# Autodesk Inventor assembly: Lidar Sensor Lexan Assembly
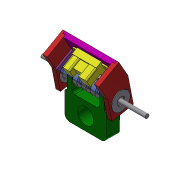
[picture p0: Inventor's stored thumbnail of the model, 180x180]
Saved by Autodesk Inventor 2018.3 (Build 223284000, 284)
## iProperties
Created: 2019-02-26
Part Number: Lidar Sensor Lexan Assembly
Document SubType Name: Assembly
Designer: aye06091
Mass: 65.9637 g
Surface Area: 342.343 cm^2
Volume: 65.9637 cm^3
Density: 1 g/cm^3
Author: aye06091
## Documents named in this file (10)
- Y:\DeSimony-R\Senior R&D\4 R&D Shared Folder\VisiStick\VisiStick (Inventor)\Case Final\Lidar Sensor Lexan Assembly.iam
- Y:\DeSimony-R\Senior R&D\4 R&D Shared Folder\VisiStick\VisiStick (Inventor)\Case Final\Lidar Sensor CAse Piece 1.ipt
- Y:\DeSimony-R\Senior R&D\4 R&D Shared Folder\VisiStick\VisiStick (Inventor)\Case Final\Lidar Sensor Case Piece 2.ipt
- Y:\DeSimony-R\Senior R&D\4 R&D Shared Folder\VisiStick\VisiStick (Inventor)\Case Final\Lidar Sensor Case Piece 3.ipt
- Y:\DeSimony-R\Senior R&D\4 R&D Shared Folder\VisiStick\VisiStick (Inventor)\Electronics\Sharp 2Y0A02.ipt
- Y:\DeSimony-R\Senior R&D\4 R&D Shared Folder\VisiStick\VisiStick (Inventor)\Physical Parts\Lidar Sensor Case 4 v2.ipt
- Y:\DeSimony-R\Senior R&D\4 R&D Shared Folder\VisiStick\VisiStick (Inventor)\Case Final\Ball Bearing.ipt
- Y:\DeSimony-R\Senior R&D\4 R&D Shared Folder\VisiStick\VisiStick (Inventor)\Case Final\Steel Rod.ipt
- Y:\DeSimony-R\Senior R&D\4 R&D Shared Folder\VisiStick\VisiStick (Inventor)\Case Final\Needle Bearing Mount v2.ipt
- Y:\DeSimony-R\Senior R&D\4 R&D Shared Folder\VisiStick\VisiStick (Inventor)\Physical Parts\T-Spacer .125 inch bore.ipt
## Components (14 placed, 9 different names)
1. Sharp 2Y0A02:1 — Insert:5, Insert:6
2. Lidar Sensor CAse Piece 1:1 — Flush:1, Flush:2, Mate:3, Insert:10
3. Lidar Sensor Case Piece 2:1 — Flush:1, Flush:2, Mate:1, Mate:2, Flush:3, Mate:4, Flush:4, Mate:5, Insert:9
4. Ball Bearing:1 — Insert:9
5. Ball Bearing:2 — Insert:10, Insert:11
6. Steel Rod:1 — Insert:11, Insert:12
7. Lidar Sensor Case 4 v2:1 — Mate:4, Flush:4, Mate:5
8. Lidar Sensor Case Piece 3:1 — Mate:1, Mate:2, Mate:3, Flush:3, Insert:5, Insert:6
9. Needle Bearing Mount v2:1 — Insert:12, Insert:13, Insert:14, Insert:15
10. T-Spacer .125 inch bore:1 — Insert:15, Insert:16
11. T-Spacer .125 inch bore:2 — Insert:14
12. T-Spacer .125 inch bore:3 — Insert:13
13. T-Spacer .125 inch bore:4 — Insert:16, Insert:17
14. T-Spacer .125 inch bore:5 — Insert:17
## Relationships (20: Insert 11, Mate 5, Flush 4)
- Flush:1: Lidar Sensor CAse Piece 1:1 ↔ Lidar Sensor Case Piece 2:1
- Flush:2: Lidar Sensor CAse Piece 1:1 ↔ Lidar Sensor Case Piece 2:1
- Mate:1: Lidar Sensor Case Piece 2:1 ↔ Lidar Sensor Case Piece 3:1
- Mate:2: Lidar Sensor Case Piece 2:1 ↔ Lidar Sensor Case Piece 3:1
- Mate:3: Lidar Sensor CAse Piece 1:1 ↔ Lidar Sensor Case Piece 3:1
- Flush:3: Lidar Sensor Case Piece 2:1 ↔ Lidar Sensor Case Piece 3:1
- Mate:4: Lidar Sensor Case Piece 2:1 ↔ Lidar Sensor Case 4 v2:1
- Flush:4: Lidar Sensor Case Piece 2:1 ↔ Lidar Sensor Case 4 v2:1
- Mate:5: Lidar Sensor Case Piece 2:1 ↔ Lidar Sensor Case 4 v2:1
- Insert:5: Sharp 2Y0A02:1 ↔ Lidar Sensor Case Piece 3:1
- Insert:6: Sharp 2Y0A02:1 ↔ Lidar Sensor Case Piece 3:1
- Insert:9: Lidar Sensor Case Piece 2:1 ↔ Ball Bearing:1
- Insert:10: Lidar Sensor CAse Piece 1:1 ↔ Ball Bearing:2
- Insert:11 (31.75 mm): Ball Bearing:2 ↔ Steel Rod:1
- Insert:12 (-37.7825 mm): Steel Rod:1 ↔ Needle Bearing Mount v2:1
- Insert:13 (0.3175 mm): Needle Bearing Mount v2:1 ↔ T-Spacer .125 inch bore:3
- Insert:14 (0.254 mm): Needle Bearing Mount v2:1 ↔ T-Spacer .125 inch bore:2
- Insert:15 (0.3175 mm): Needle Bearing Mount v2:1 ↔ T-Spacer .125 inch bore:1
- Insert:16: T-Spacer .125 inch bore:1 ↔ T-Spacer .125 inch bore:4
- Insert:17: T-Spacer .125 inch bore:4 ↔ T-Spacer .125 inch bore:5
